# Autodesk Inventor assembly: robot
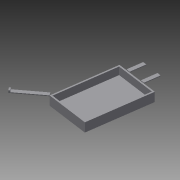
[picture p0: Inventor's stored thumbnail of the model, 180x180]
Saved by Autodesk Inventor 2015 (Build 190159000, 159)
## iProperties
Created: 2015-01-07
Part Number: robot
Document SubType Name: Assembly
Designer: harrykuperstein
Author: harrykuperstein
## Documents named in this file (4)
- C:\Users\harrykuperstein\Documents\Inventor\Content Center Files\R2015\robot.iam
- C:\Users\harrykuperstein\Documents\Inventor\Content Center Files\R2015\travel base.ipt
- C:\Users\harrykuperstein\Documents\Inventor\Content Center Files\R2015\hook.ipt
- C:\Users\harrykuperstein\Documents\Inventor\Content Center Files\R2015\half hook.ipt
## Components (9 placed, 3 different names)
1. travel base:1 — Mate:1, Mate:2, Mate:3, Mate:4, Flush:11, Rotational:1
2. hook:1 — Flush:12, Mate:10, Flush:13
3. half hook:1 — Flush:9, Flush:10, Mate:9, Flush:12, Mate:10, Flush:13
4. half hook:2 — Flush:7, Flush:8, Mate:7, Flush:11, Rotational:1
5. half hook:3 — Flush:1, Flush:2, Mate:5
6. half hook:4 — Mate:2, Mate:4, Flush:1, Flush:2, Mate:5
7. half hook:5 — Mate:1, Mate:3, Flush:3, Flush:4, Flush:5, Mate:6
8. half hook:6 — Flush:3, Flush:4, Flush:5, Mate:6
9. half hook:7 — Flush:7, Flush:8, Mate:7, Flush:9, Flush:10, Mate:9
## Relationships (22: Flush 12, Mate 9, RevoluteJoint 1)
- Mate:1: travel base:1 ↔ half hook:5
- Mate:2: travel base:1 ↔ half hook:4
- Mate:3: travel base:1 ↔ half hook:5
- Mate:4: travel base:1 ↔ half hook:4
- Flush:1: half hook:3 ↔ half hook:4
- Flush:2: half hook:3 ↔ half hook:4
- Flush:3: half hook:5 ↔ half hook:6
- Flush:4: half hook:5 ↔ half hook:6
- Flush:5: half hook:5 ↔ half hook:6
- Mate:5: half hook:3 ↔ half hook:4
- Mate:6: half hook:5 ↔ half hook:6
- Flush:7: half hook:2 ↔ half hook:7
- Flush:8: half hook:2 ↔ half hook:7
- Mate:7: half hook:2 ↔ half hook:7
- Flush:9: half hook:1 ↔ half hook:7
- Flush:10: half hook:1 ↔ half hook:7
- Mate:9: half hook:1 ↔ half hook:7
- Flush:11: travel base:1 ↔ half hook:2
- Rotational:1 [RevoluteJoint]: travel base:1 ↔ half hook:2
- Flush:12: hook:1 ↔ half hook:1
- Mate:10: hook:1 ↔ half hook:1
- Flush:13: hook:1 ↔ half hook:1
